# Autodesk Inventor assembly: Ensamblaje1
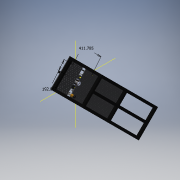
[picture p0: Inventor's stored thumbnail of the model, 180x180]
Saved by Autodesk Inventor 2018 (Build 220112000, 112)
## iProperties
Created: 2017-11-04
Part Number: Ensamblaje1
Material: Genérico
Document SubType Name: Assembly
Designer: Andres
Author: Andres
## Documents named in this file (4)
- C:\Users\Andres\Documents\MOT\sistema_completo\Ensamblaje1.iam
- C:\Users\Andres\Documents\MOT\ensamblaje_inventor\Ensamblaje_MOT.iam
- C:\Users\Andres\Documents\MOT\Zeeman\ensamblaje\Bobina_grande.iam
- C:\Users\Andres\Documents\MOT\partes\base_sistema\Pieza57.ipt
## Components (5 placed, 3 different names)
1. Ensamblaje_MOT:1 [sub-assembly] — De rotación:1
2. Bobina_grande:1 [sub-assembly] — De rotación:1, De rotación:2, De rotación:3, De rotación:4
3. Pieza57:1 — De rotación:4
4. Pieza57:2 — De rotación:2
5. Pieza57:3 — De rotación:3
## Relationships (4: RevoluteJoint 4)
- De rotación:1 [RevoluteJoint]: Ensamblaje_MOT:1 ↔ Bobina_grande:1
- De rotación:2 [RevoluteJoint]: Bobina_grande:1 ↔ Pieza57:2
- De rotación:3 [RevoluteJoint]: Bobina_grande:1 ↔ Pieza57:3
- De rotación:4 [RevoluteJoint]: Bobina_grande:1 ↔ Pieza57:1
